# Autodesk Inventor assembly: head
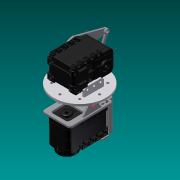
[picture p0: Inventor's stored thumbnail of the model, 180x180]
Saved by Autodesk Inventor 2013 SP2 (Build 170200200, 200)
## iProperties
Created: 2014-11-25
Part Number: head
Document SubType Name: Assembly
Designer: Master
Author: Master
## Documents named in this file (6)
- C:\Users\Master\Documents\GitHub\DIY-HR-OS1\CAD Files\head.iam
- C:\Users\Master\Documents\GitHub\DIY-HR-OS1\CAD Files\AX12\AX12.iam
- C:\Users\Master\Documents\GitHub\DIY-HR-OS1\CAD Files\headtilt-teardrop.ipt
- C:\Users\Master\Documents\GitHub\DIY-HR-OS1\CAD Files\headtilt-long.ipt
- C:\Users\Master\Documents\GitHub\DIY-HR-OS1\CAD Files\head-mount.ipt
- C:\Users\Master\Documents\GitHub\DIY-HR-OS1\CAD Files\headtilt-base2.ipt
## Components (6 placed, 5 different names)
1. AX12:1 [sub-assembly] — Mate:1, Mate:2, Mate:3, Mate:4, Flush:1, Flush:2, Flush:3
2. headtilt-teardrop:1 — Mate:3, Mate:4, Mate:5, Mate:6
3. headtilt-long:1 — Mate:5, Mate:6, Mate:10
4. head-mount:1 — Flush:1, Flush:2, Flush:3, Mate:8, Mate:9
5. AX12:2 [sub-assembly] — Mate:7
6. headtilt-base2:1 — Mate:7, Mate:8, Mate:9, Mate:10
## Relationships (13: Mate 10, Flush 3)
- Mate:1: AX12:1
- Mate:2: AX12:1
- Mate:3: AX12:1 ↔ headtilt-teardrop:1
- Mate:4: AX12:1 ↔ headtilt-teardrop:1
- Mate:5: headtilt-teardrop:1 ↔ headtilt-long:1
- Mate:6: headtilt-teardrop:1 ↔ headtilt-long:1
- Flush:1: AX12:1 ↔ head-mount:1
- Flush:2: AX12:1 ↔ head-mount:1
- Flush:3: AX12:1 ↔ head-mount:1
- Mate:7: AX12:2 ↔ headtilt-base2:1
- Mate:8: head-mount:1 ↔ headtilt-base2:1
- Mate:9: head-mount:1 ↔ headtilt-base2:1
- Mate:10: headtilt-long:1 ↔ headtilt-base2:1
